# Autodesk Inventor assembly: Cl1-100
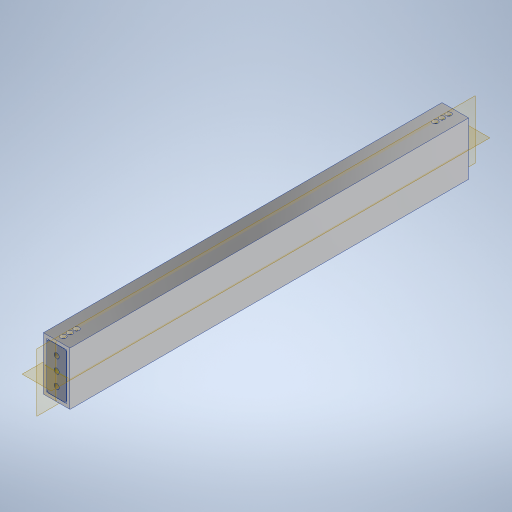
[picture p0: Inventor's stored thumbnail of the model, 512x512]
Saved by Autodesk Inventor 2023.4 (Build 274418000, 418)
## iProperties
Created: 2025-01-18
Part Number: Cl1-100
Document SubType Name: Assembly
Designer: mavericks
Author: mavericks
## Documents named in this file (3)
- C:\Users\mavericks\Documents\Robotics\GitHub\2025-ReefScape---CAD\Climber\Cl1-100.iam
- C:\Users\mavericks\Documents\Robotics\GitHub\2025-ReefScape---CAD\Climber\Cl1-003.ipt
- C:\Users\mavericks\Documents\Robotics\GitHub\2025-ReefScape---CAD\Climber\CL1-004.ipt
## Components (3 placed, 2 different names)
1. CL1-004:1 — Mate:1, Flush:1, Mate:2, Flush:2
2. CL1-004:2 — Flush:3, Mate:3, Mate:4
3. Cl1-003:1 — Mate:1, Flush:1, Mate:2, Flush:2, Flush:3, Mate:3, Mate:4
## Relationships (7: Mate 4, Flush 3)
- Mate:1: CL1-004:1 ↔ Cl1-003:1
- Flush:1: CL1-004:1 ↔ Cl1-003:1
- Mate:2: CL1-004:1 ↔ Cl1-003:1
- Flush:2: CL1-004:1 ↔ Cl1-003:1
- Flush:3: CL1-004:2 ↔ Cl1-003:1
- Mate:3: CL1-004:2 ↔ Cl1-003:1
- Mate:4: CL1-004:2 ↔ Cl1-003:1
